# Autodesk Inventor assembly: Optics Assembly Window
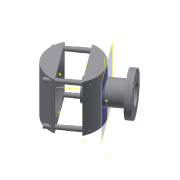
[picture p0: Inventor's stored thumbnail of the model, 180x180]
Saved by Autodesk Inventor 2015 (Build 190159000, 159)
## iProperties
Created: 2014-07-17
Part Number: Optics Assembly Window
Document SubType Name: Assembly
Designer: I Rabey
Author: I Rabey
## Documents named in this file (7)
- C:\CADFiles\EDM Machine\Detection Region\Re-entrant Flange and Mirrors\Optics Assembly Window.iam
- C:\CADFiles\EDM Machine\Detection Region\Re-entrant Flange and Mirrors\Mirrors\Ideas\Mirror Assembly.iam
- C:\CADFiles\EDM Machine\Detection Region\Re-entrant Flange and Mirrors\Mirrors\Custom Mirror Design.ipt
- C:\CADFiles\EDM Machine\Detection Region\Re-entrant Flange and Mirrors\Mirrors\Custom Mirror Design Part 2.ipt
- C:\CADFiles\EDM Machine\Detection Region\Re-entrant Flange and Mirrors\holdingRod.ipt
- C:\CADFiles\EDM Machine\Detection Region\Re-entrant Flange and Mirrors\Re-entrant Flange window.iam
- C:\CADFiles\EDM Machine\Detection Region\Re-entrant Flange and Mirrors\retainingring.ipt
## Components (9 placed, 6 different names)
1. Mirror Assembly:1 [sub-assembly]
2. Custom Mirror Design:1 — Mate:31, Mate:32
3. Custom Mirror Design Part 2:1 — Mate:27, Insert:1, Insert:2, Insert:3, Mate:29, Angle:1, Mate:32, Mate:35, Mate:36, Mate:38
4. holdingRod:1 — Insert:3
5. holdingRod:2 — Insert:1, Mate:31
6. holdingRod:3 — Insert:2
7. holdingRod:4 — Mate:29
8. Re-entrant Flange window:1 [sub-assembly] — Mate:35, Mate:36, Mate:37
9. retainingring:1 — Mate:37, Mate:38
## Relationships (14: Mate 10, Insert 3, Angle 1)
- Mate:11
- Mate:12
- Mate:27 (75 mm): Custom Mirror Design Part 2:1
- Insert:1: Custom Mirror Design Part 2:1 ↔ holdingRod:2
- Insert:2: Custom Mirror Design Part 2:1 ↔ holdingRod:3
- Insert:3: Custom Mirror Design Part 2:1 ↔ holdingRod:1
- Mate:29: Custom Mirror Design Part 2:1 ↔ holdingRod:4
- Mate:31: Custom Mirror Design:1 ↔ holdingRod:2
- Angle:1 (0 deg): Custom Mirror Design Part 2:1
- Mate:32 (59.4 mm): Custom Mirror Design:1 ↔ Custom Mirror Design Part 2:1
- Mate:35: Custom Mirror Design Part 2:1 ↔ Re-entrant Flange window:1
- Mate:36: Custom Mirror Design Part 2:1 ↔ Re-entrant Flange window:1
- Mate:37: Re-entrant Flange window:1 ↔ retainingring:1
- Mate:38: Custom Mirror Design Part 2:1 ↔ retainingring:1
